# Autodesk Inventor assembly: Mantis Blade assembly (This fuckass assembly took so goddamn long and it really sucks because inventor is a less than favorable squared of a program AHHHHHHHH)
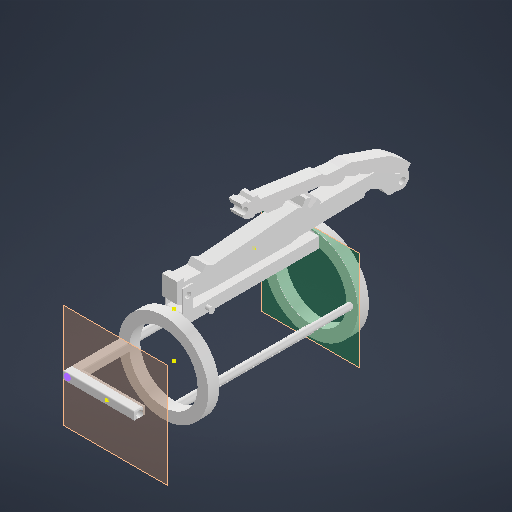
[picture p0: Inventor's stored thumbnail of the model, 512x512]
Saved by Autodesk Inventor 2025.2 (Build 292293000, 293)
## iProperties
Created: 2025-04-09
Part Number: Mantis Blade assembly (This fuckass assembly took so goddamn long and it really sucks because inventor is a less than favorable squared of a program AHHHHHHHH)
Document SubType Name: Assembly
Designer: Jameson Huang
Author: Jameson Huang
## Documents named in this file (4)
- C:\Users\Jameson Huang\Downloads\Mantis Blade assembly (This fuckass assembly took so goddamn long and it really sucks because inventor is a less than favorable squared of a program AHHHHHHHH).iam
- C:\Users\Jameson Huang\Downloads\Capstone Arm Brace 2.ipt
- C:\Users\Jameson Huang\Downloads\Scale Connector.ipt
- C:\Users\Jameson Huang\Downloads\Blade slider.ipt
## Components (3 placed, 3 different names)
1. Capstone Arm Brace 2:1 — Mate:1
2. Scale Connector:2 — Mate:1, Mate:2
3. Blade slider:1 — Mate:2
## Relationships (2: Mate 2)
- Mate:1: Capstone Arm Brace 2:1 ↔ Scale Connector:2
- Mate:2: Scale Connector:2 ↔ Blade slider:1
